# Autodesk Inventor assembly: Montagem Completa
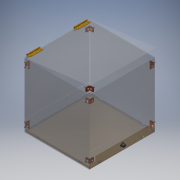
[picture p0: Inventor's stored thumbnail of the model, 180x180]
Saved by Autodesk Inventor 2018 (Build 220112000, 112)
## iProperties
Created: 2018-07-09
Part Number: Montagem Completa
Material: Genérico
Document SubType Name: Assembly
Designer: Regner
Author: Regner
## Documents named in this file (6)
- C:\Users\Regner\Documents\ROBOTA\2018\Tortura Ratos\Montagem Completa.iam
- C:\Users\Regner\Documents\ROBOTA\2018\Tortura Ratos\Gaveta.iam
- C:\Users\Regner\Documents\ROBOTA\2018\Tortura Ratos\Montagem Lateral.iam
- C:\Users\Regner\Documents\ROBOTA\2018\Tortura Ratos\012894_a.ipt
- C:\Users\Regner\Documents\ROBOTA\2018\Tortura Ratos\012895_b.ipt
- C:\Users\Regner\Documents\ROBOTA\2018\Tortura Ratos\Tampa.ipt
## Components (7 placed, 5 different names)
1. Gaveta:1 [sub-assembly] — Coincidência:1, Alinhamento:1, Alinhamento:2, Alinhamento:3, Alinhamento:4, Alinhamento:5
2. Montagem Lateral:1 [sub-assembly] — Coincidência:1, Alinhamento:1, Alinhamento:2, Coincidência:6, Alinhamento:6, Alinhamento:7, Coincidência:7, Alinhamento:8, Alinhamento:9
3. DIV / Schanier / 012894.ipt / Schanier:1 — Coincidência:2, Coincidência:4, Coincidência:7, Alinhamento:8, Alinhamento:9
4. DIV / Schanier / 012895.ipt / Schanier B-Seite:1 — Coincidência:2, Coincidência:4, Coincidência:9, Alinhamento:11
5. DIV / Schanier / 012894.ipt / Schanier:2 — Coincidência:3, Coincidência:5, Coincidência:6, Alinhamento:6, Alinhamento:7
6. DIV / Schanier / 012895.ipt / Schanier B-Seite:2 — Coincidência:3, Coincidência:5, Coincidência:8, Alinhamento:10
7. Tampa:1 — Coincidência:8, Coincidência:9, Alinhamento:10, Alinhamento:11
## Relationships (20: Flush 11, Mate 9)
- Coincidência:1 [Mate]: Gaveta:1 ↔ Montagem Lateral:1
- Alinhamento:1 [Flush]: Gaveta:1 ↔ Montagem Lateral:1
- Alinhamento:2 [Flush]: Gaveta:1 ↔ Montagem Lateral:1
- Alinhamento:3 [Flush]: Gaveta:1
- Alinhamento:4 [Flush]: Gaveta:1
- Alinhamento:5 [Flush]: Gaveta:1
- Coincidência:2 [Mate]: DIV / Schanier / 012894.ipt / Schanier:1 ↔ DIV / Schanier / 012895.ipt / Schanier B-Seite:1
- Coincidência:3 [Mate]: DIV / Schanier / 012894.ipt / Schanier:2 ↔ DIV / Schanier / 012895.ipt / Schanier B-Seite:2
- Coincidência:4 [Mate]: DIV / Schanier / 012894.ipt / Schanier:1 ↔ DIV / Schanier / 012895.ipt / Schanier B-Seite:1
- Coincidência:5 [Mate]: DIV / Schanier / 012894.ipt / Schanier:2 ↔ DIV / Schanier / 012895.ipt / Schanier B-Seite:2
- Coincidência:6 [Mate]: Montagem Lateral:1 ↔ DIV / Schanier / 012894.ipt / Schanier:2
- Alinhamento:6 [Flush]: Montagem Lateral:1 ↔ DIV / Schanier / 012894.ipt / Schanier:2
- Alinhamento:7 [Flush] (10 mm): Montagem Lateral:1 ↔ DIV / Schanier / 012894.ipt / Schanier:2
- Coincidência:7 [Mate]: Montagem Lateral:1 ↔ DIV / Schanier / 012894.ipt / Schanier:1
- Alinhamento:8 [Flush]: Montagem Lateral:1 ↔ DIV / Schanier / 012894.ipt / Schanier:1
- Alinhamento:9 [Flush] (10 mm): Montagem Lateral:1 ↔ DIV / Schanier / 012894.ipt / Schanier:1
- Coincidência:8 [Mate]: DIV / Schanier / 012895.ipt / Schanier B-Seite:2 ↔ Tampa:1
- Coincidência:9 [Mate]: DIV / Schanier / 012895.ipt / Schanier B-Seite:1 ↔ Tampa:1
- Alinhamento:10 [Flush] (5 mm): DIV / Schanier / 012895.ipt / Schanier B-Seite:2 ↔ Tampa:1
- Alinhamento:11 [Flush] (15 mm): DIV / Schanier / 012895.ipt / Schanier B-Seite:1 ↔ Tampa:1
